# Autodesk Inventor assembly: seguidor_speed
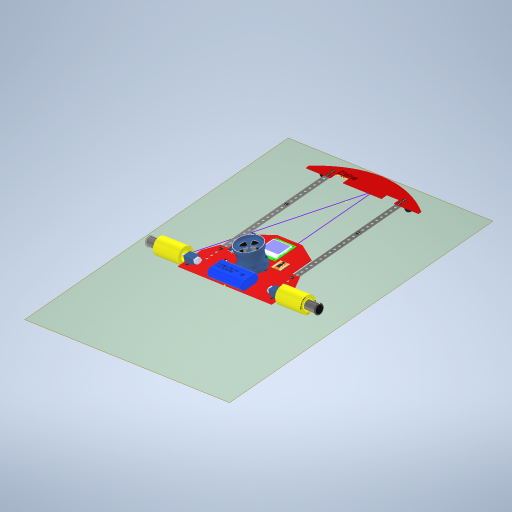
[picture p0: Inventor's stored thumbnail of the model, 512x512]
Saved by Autodesk Inventor 2023 (Build 270158000, 158)
## iProperties
Created: 2023-08-07
Part Number: seguidor_speed
Document SubType Name: Assembly
Designer: azeve
Author: azeve
## Documents named in this file (21)
- C:\Users\azeve\OneDrive\Área de Trabalho\seguidor_linha\seguidor_speed.iam
- C:\Users\azeve\OneDrive\Área de Trabalho\seguidor_linha\Peça3.ipt
- C:\Users\azeve\OneDrive\Área de Trabalho\seguidor_linha\aste.ipt
- C:\Users\azeve\OneDrive\Área de Trabalho\seguidor_linha\esfera.ipt
- C:\Users\azeve\OneDrive\Área de Trabalho\seguidor_linha\acoplamento_esfera.ipt
- C:\Users\azeve\OneDrive\Área de Trabalho\cad_seguidor\Peças GrabCad\n20-motor-1.snapshot.1\N20 Motor.ipt
- C:\Users\azeve\OneDrive\Área de Trabalho\cad_seguidor\Peças GrabCad\sparkfun-motor-driver-dual-tb6612fng-1a-1.snapshot.5\Motor Driver.ipt
- C:\Users\azeve\OneDrive\Área de Trabalho\cad_seguidor\Peças GrabCad\stm32f103c8t6-board-1.snapshot.2\stm32f103c8t6-board.ipt
- C:\Users\azeve\OneDrive\Área de Trabalho\cad_seguidor\Peças GrabCad\nokia-5110-1.snapshot.1\Nokia 5110.ipt
- C:\Users\azeve\OneDrive\Área de Trabalho\cad_seguidor\Peças GrabCad\2S 7,4V 1500 mAh Battery.ipt
- C:\Users\azeve\OneDrive\Área de Trabalho\seguidor_linha\acoplament_ventoinha.ipt
- C:\Users\azeve\OneDrive\Área de Trabalho\seguidor_linha\acompletado_vetoinha.ipt
- C:\Users\azeve\OneDrive\Área de Trabalho\seguidor_linha\acoplamento_ventoinha1.ipt
- C:\Users\azeve\OneDrive\Área de Trabalho\seguidor_linha\roda.ipt
- C:\Users\azeve\OneDrive\Área de Trabalho\seguidor_linha\pneu.ipt
- C:\Users\azeve\OneDrive\Área de Trabalho\seguidor_linha\sensores1.ipt
- C:\Users\azeve\OneDrive\Área de Trabalho\seguidor_linha\parafusos.ipt
- C:\Users\azeve\OneDrive\Área de Trabalho\seguidor_linha\engate_motor.ipt
- C:\Users\azeve\OneDrive\Área de Trabalho\seguidor_linha\prafuso3.ipt
- C:\Users\azeve\OneDrive\Área de Trabalho\seguidor_linha\motor_ven.ipt
- C:\Users\azeve\OneDrive\Área de Trabalho\seguidor_linha\helice.ipt
## Components (42 placed, 20 different names)
1. Peça3:1 — Inserir:3, Inserir:4, Coincidente:3, Coincidente:4, Coincidente:5, Coincidente:6, Coincidente:8, Rotativa:1, Rotativa:2, Alinhado:1, Rotativa:20, Rotativa:21, Alinhado:2
2. aste:1 — Inserir:4, Coincidente:9, Rotativa:15
3. aste:2 — Inserir:3, Rotativa:14
4. esfera:1 — Tangente:1
5. esfera:2 — Tangente:2
6. acoplamento_esfera:1 — Tangente:1
7. acoplamento_esfera:2 — Tangente:2
8. N20 Motor:2 — Coincidente:3, Inserir:7, Coincidente:12
9. Motor Driver:1 — Coincidente:4
10. stm32f103c8t6-board:1
11. Nokia 5110:1 — Coincidente:5
12. N20 Motor:3 — Coincidente:6, Inserir:8, Coincidente:13
13. 2S 7,4V 1500 mAh Battery:1 — Coincidente:8
14. acoplament_ventoinha:1 — Rotativa:1
15. acompletado_vetoinha:1
16. acoplamento_ventoinha1:1 — Rotativa:2, Rotativa:7, Rígida:1, Rotativa:22, Rotativa:23, Rotativa:24
17. roda:1 — Inserir:5, Inserir:7
18. roda:2 — Inserir:6, Inserir:8
19. pneu:1 — Inserir:5
20. pneu:2 — Inserir:6
21. sensores1:1 — Coincidente:9, Rotativa:16, Rotativa:17, Rotativa:18, Rotativa:19
22. parafusos:7 — Rotativa:14
23. engate_motor:1 — Coincidente:12, Rotativa:8, Rotativa:9
24. engate_motor:2 — Coincidente:13, Rotativa:10, Rotativa:11
25. prafuso3:1 — Rígida:1
26. prafuso3:2 — Rotativa:7
27. prafuso3:3 — Rotativa:10
28. prafuso3:4 — Rotativa:11
29. prafuso3:5 — Rotativa:8
30. prafuso3:6 — Rotativa:9
31. parafusos:10 — Rotativa:15
32. parafusos:11 — Rotativa:21
33. parafusos:12 — Rotativa:19
34. parafusos:13 — Rotativa:17
35. parafusos:14 — Rotativa:16
36. parafusos:15 — Rotativa:18
37. parafusos:16 — Rotativa:20
38. motor_ven:1 — Rotativa:22, Coincidente:14
39. helice:1 — Coincidente:14
40. prafuso3:7
41. prafuso3:10 — Rotativa:24
42. prafuso3:11 — Rotativa:23
## Relationships (38: RevoluteJoint 18, Mate 9, Insert 6, Tangent 2, Flush 2, WeldJoint 1)
- Tangente:1: esfera:1 ↔ acoplamento_esfera:1
- Tangente:2: esfera:2 ↔ acoplamento_esfera:2
- Inserir:3: Peça3:1 ↔ aste:2
- Inserir:4: Peça3:1 ↔ aste:1
- Coincidente:3 [Mate]: Peça3:1 ↔ N20 Motor:2
- Coincidente:4 [Mate]: Peça3:1 ↔ Motor Driver:1
- Coincidente:5 [Mate]: Peça3:1 ↔ Nokia 5110:1
- Coincidente:6 [Mate]: Peça3:1 ↔ N20 Motor:3
- Coincidente:8 [Mate]: Peça3:1 ↔ 2S 7,4V 1500 mAh Battery:1
- Rotativa:1 [RevoluteJoint]: Peça3:1 ↔ acoplament_ventoinha:1
- Rotativa:2 [RevoluteJoint]: Peça3:1 ↔ acoplamento_ventoinha1:1
- Inserir:5: roda:1 ↔ pneu:1
- Inserir:6: roda:2 ↔ pneu:2
- Inserir:7: N20 Motor:2 ↔ roda:1
- Inserir:8: N20 Motor:3 ↔ roda:2
- Coincidente:9 [Mate]: aste:1 ↔ sensores1:1
- Coincidente:12 [Mate]: N20 Motor:2 ↔ engate_motor:1
- Coincidente:13 [Mate]: N20 Motor:3 ↔ engate_motor:2
- Rotativa:7 [RevoluteJoint]: acoplamento_ventoinha1:1 ↔ prafuso3:2
- Rígida:1 [WeldJoint]: acoplamento_ventoinha1:1 ↔ prafuso3:1
- Alinhado:1 [Flush]: Peça3:1
- Rotativa:8 [RevoluteJoint]: engate_motor:1 ↔ prafuso3:5
- Rotativa:9 [RevoluteJoint]: engate_motor:1 ↔ prafuso3:6
- Rotativa:10 [RevoluteJoint]: engate_motor:2 ↔ prafuso3:3
- Rotativa:11 [RevoluteJoint]: engate_motor:2 ↔ prafuso3:4
- Rotativa:14 [RevoluteJoint]: aste:2 ↔ parafusos:7
- Rotativa:15 [RevoluteJoint]: aste:1 ↔ parafusos:10
- Rotativa:16 [RevoluteJoint]: sensores1:1 ↔ parafusos:14
- Rotativa:17 [RevoluteJoint]: sensores1:1 ↔ parafusos:13
- Rotativa:18 [RevoluteJoint]: sensores1:1 ↔ parafusos:15
- Rotativa:19 [RevoluteJoint]: sensores1:1 ↔ parafusos:12
- Rotativa:20 [RevoluteJoint]: Peça3:1 ↔ parafusos:16
- Rotativa:21 [RevoluteJoint]: Peça3:1 ↔ parafusos:11
- Rotativa:22 [RevoluteJoint]: acoplamento_ventoinha1:1 ↔ motor_ven:1
- Coincidente:14 [Mate]: motor_ven:1 ↔ helice:1
- Rotativa:23 [RevoluteJoint]: acoplamento_ventoinha1:1 ↔ prafuso3:11
- Rotativa:24 [RevoluteJoint]: acoplamento_ventoinha1:1 ↔ prafuso3:10
- Alinhado:2 [Flush] (12.75 mm): Peça3:1
